# Autodesk Inventor assembly: Anbindung test-Inventor
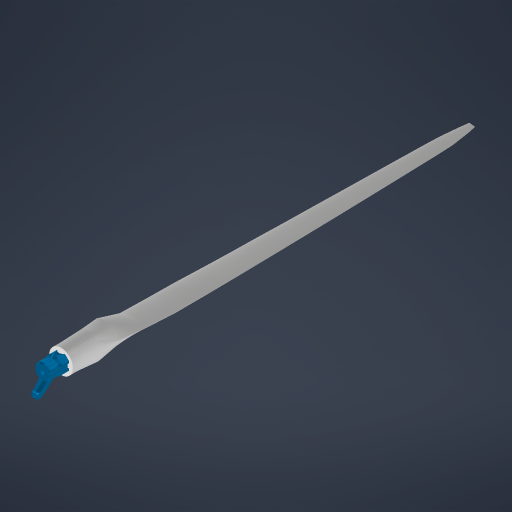
[picture p0: Inventor's stored thumbnail of the model, 512x512]
Saved by Autodesk Inventor 2023.2 (Build 272271000, 271)
## iProperties
Created: 2023-04-05
Part Number: Anbindung test-Inventor
Document SubType Name: Assembly
Designer: tadeus
Author: tadeus
## Documents named in this file (3)
- C:\Users\tadeu\Documents\0 Nerdy\CAD\Inventor\Studium\5. Semester\NWPL\WKA\Anbindung test-Inventor.iam
- C:\Users\tadeu\Documents\0 Nerdy\CAD\Inventor\Studium\5. Semester\NWPL\WKA\RotorArm.ipt
- C:\Users\tadeu\Ts Programme\Studium\NREL5MW\5MW_6X.ipt
## Components (2 placed, 2 different names)
1. RotorArm:1 — Einfügen:1
2. 5MW_6X:1 — Einfügen:1
## Relationships (1: Insert 1)
- Einfügen:1 [Insert] (-16 mm): RotorArm:1 ↔ 5MW_6X:1
